# Autodesk Inventor assembly: ttest
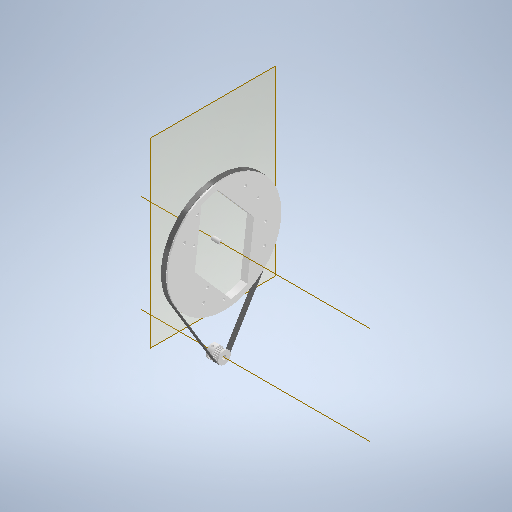
[picture p0: Inventor's stored thumbnail of the model, 512x512]
Saved by Autodesk Inventor 2025.1 (Build 291241020, 241B)
## iProperties
Created: 2025-05-16
Part Number: ttest
Document SubType Name: Assembly
Designer: tiago
Author: tiago
## Documents named in this file (6)
- C:\Users\tiago\Documents\Inventor\SCRA\ttest.iam
- C:\Users\tiago\Documents\Inventor\SCRA\GT2Pulley_z220.ipt
- GT2Pulley_z220.ipt
- C:\Users\tiago\Documents\Inventor\SCRA\GT2Pulley_z20.ipt
- C:\Users\tiago\Documents\Inventor\SCRA\PontoTest.ipt
- C:\Users\tiago\Documents\Inventor\SCRA\ttest\Design Accelerator\Synchronous Belts Transmission3.iam
## Components (4 placed, 4 different names)
1. GT2Pulley_z220:1 — Mate:1, Flush:4, Rotation:1
2. GT2Pulley_z20:1 — Mate:2, Flush:3, Rotation:1
3. PontoTest:1 — Flush:1, Flush:2, Mate:1, Mate:2, Flush:3, Flush:4
4. Synchronous Belts Transmission:1 [sub-assembly]
## Relationships (7: Flush 4, Mate 2, RelateRotation 1)
- Flush:1: PontoTest:1
- Flush:2: PontoTest:1
- Mate:1: GT2Pulley_z220:1 ↔ PontoTest:1
- Mate:2: GT2Pulley_z20:1 ↔ PontoTest:1
- Flush:3 (5 mm): GT2Pulley_z20:1 ↔ PontoTest:1
- Flush:4 (5 mm): GT2Pulley_z220:1 ↔ PontoTest:1
- Rotation:1 [RelateRotation] (1 ul): GT2Pulley_z220:1 ↔ GT2Pulley_z20:1
